# Autodesk Inventor assembly: CC2x2
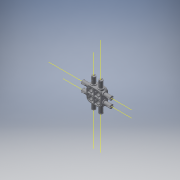
[picture p0: Inventor's stored thumbnail of the model, 180x180]
Saved by Autodesk Inventor 2019.3 (Build 233278000, 278)
## iProperties
Created: 2019-02-06
Part Number: CC2x2
Document SubType Name: Assembly
Designer: Varga Daniel
Author: Varga Daniel
## Documents named in this file (5)
- C:\!_Dani\!_cloud\OneDrive\!_munka\Revolution\RevvyDemoKit\Structural parts\Connector Boxes\Connector cubes\CC2x2_X.iam
- C:\!_Dani\!_cloud\OneDrive\!_munka\Revolution\RevvyDemoKit\Structural parts\Connector Boxes\Connector_box_L_base.ipt
- C:\!_Dani\!_cloud\OneDrive\!_munka\Revolution\RevvyDemoKit\Structural parts\Connector Boxes\Connector_box_collar\Connector_box_collar-one_side.ipt
- C:\!_Dani\!_cloud\OneDrive\!_munka\Revolution\RevvyDemoKit\Structural parts\Connector Boxes\Connector_box_collar.ipt
- C:\!_Dani\!_cloud\OneDrive\!_munka\Revolution\RevvyDemoKit\Structural parts\Connetor Pins\Connector_pin_stick.ipt
## Components (20 placed, 3 different names)
1. Connector_box_L_base:1 — Flush:1, Flush:2, Mate:41, Flush:3, Flush:4, Mate:42, Mate:54, Mate:55, Angle:6, Mate:56, Mate:57, Angle:7
2. Connector_box_collar-one_side:1 — Mate:7, Mate:8, Mate:57
3. Connector_box_collar-one_side:2 — Mate:9, Mate:10, Mate:55
4. Connector_pin_stick:1 — Mate:7, Mate:8, Mate:56, Angle:7
5. Connector_pin_stick:2 — Mate:9, Mate:10, Mate:54, Angle:6
6. Connector_box_collar-one_side:3 — Mate:47
7. Connector_box_collar-one_side:4 — Mate:49
8. Connector_pin_stick:3 — Mate:46, Angle:2
9. Connector_pin_stick:4 — Mate:48, Angle:3
10. Connector_box_collar-one_side:5 — Mate:51
11. Connector_box_collar-one_side:6 — Mate:53
12. Connector_pin_stick:5 — Mate:50, Angle:4
13. Connector_pin_stick:6 — Mate:52, Angle:5
14. Connector_box_collar-one_side:7 — Mate:45
15. Connector_box_collar-one_side:8 — Mate:59
16. Connector_pin_stick:7 — Mate:44, Angle:1
17. Connector_pin_stick:8 — Mate:58, Angle:8
18. Connector_box_L_base:6 — Flush:1, Flush:2, Mate:41, Flush:5, Flush:6, Mate:43, Mate:44, Mate:45, Angle:1, Mate:58, Mate:59, Angle:8
19. Connector_box_L_base:7 — Flush:3, Flush:4, Mate:42, Mate:50, Mate:51, Angle:4, Mate:52, Mate:53, Angle:5
20. Connector_box_L_base:8 — Flush:5, Flush:6, Mate:43, Mate:46, Mate:47, Angle:2, Mate:48, Mate:49, Angle:3
## Relationships (49: Mate 35, Angle 8, Flush 6)
- Mate:7: Connector_box_collar-one_side:1 ↔ Connector_pin_stick:1
- Mate:8: Connector_box_collar-one_side:1 ↔ Connector_pin_stick:1
- Mate:9: Connector_box_collar-one_side:2 ↔ Connector_pin_stick:2
- Mate:10: Connector_box_collar-one_side:2 ↔ Connector_pin_stick:2
- [Mate]: Connector_box_collar-one_side:3 ↔ Connector_pin_stick:3
- [Mate]: Connector_box_collar-one_side:3 ↔ Connector_pin_stick:3
- [Mate]: Connector_box_collar-one_side:4 ↔ Connector_pin_stick:4
- [Mate]: Connector_box_collar-one_side:4 ↔ Connector_pin_stick:4
- [Mate]: Connector_box_collar-one_side:5 ↔ Connector_pin_stick:5
- [Mate]: Connector_box_collar-one_side:5 ↔ Connector_pin_stick:5
- [Mate]: Connector_box_collar-one_side:6 ↔ Connector_pin_stick:6
- [Mate]: Connector_box_collar-one_side:6 ↔ Connector_pin_stick:6
- [Mate]: Connector_box_collar-one_side:7 ↔ Connector_pin_stick:7
- [Mate]: Connector_box_collar-one_side:7 ↔ Connector_pin_stick:7
- [Mate]: Connector_box_collar-one_side:8 ↔ Connector_pin_stick:8
- [Mate]: Connector_box_collar-one_side:8 ↔ Connector_pin_stick:8
- Flush:1: Connector_box_L_base:1 ↔ Connector_box_L_base:6
- Flush:2: Connector_box_L_base:1 ↔ Connector_box_L_base:6
- Mate:41: Connector_box_L_base:1 ↔ Connector_box_L_base:6
- Flush:3: Connector_box_L_base:1 ↔ Connector_box_L_base:7
- Flush:4: Connector_box_L_base:1 ↔ Connector_box_L_base:7
- Mate:42: Connector_box_L_base:1 ↔ Connector_box_L_base:7
- Flush:5: Connector_box_L_base:6 ↔ Connector_box_L_base:8
- Flush:6: Connector_box_L_base:6 ↔ Connector_box_L_base:8
- Mate:43: Connector_box_L_base:6 ↔ Connector_box_L_base:8
- Mate:44: Connector_pin_stick:7 ↔ Connector_box_L_base:6
- Mate:45: Connector_box_collar-one_side:7 ↔ Connector_box_L_base:6
- Angle:1 (0 deg): Connector_pin_stick:7 ↔ Connector_box_L_base:6
- Mate:46: Connector_pin_stick:3 ↔ Connector_box_L_base:8
- Mate:47: Connector_box_collar-one_side:3 ↔ Connector_box_L_base:8
- Angle:2 (0 deg): Connector_pin_stick:3 ↔ Connector_box_L_base:8
- Mate:48: Connector_pin_stick:4 ↔ Connector_box_L_base:8
- Mate:49: Connector_box_collar-one_side:4 ↔ Connector_box_L_base:8
- Angle:3 (0 deg): Connector_pin_stick:4 ↔ Connector_box_L_base:8
- Mate:50: Connector_pin_stick:5 ↔ Connector_box_L_base:7
- Mate:51: Connector_box_collar-one_side:5 ↔ Connector_box_L_base:7
- Angle:4 (0 deg): Connector_pin_stick:5 ↔ Connector_box_L_base:7
- Mate:52: Connector_pin_stick:6 ↔ Connector_box_L_base:7
- Mate:53: Connector_box_collar-one_side:6 ↔ Connector_box_L_base:7
- Angle:5 (0 deg): Connector_pin_stick:6 ↔ Connector_box_L_base:7
- Mate:54: Connector_box_L_base:1 ↔ Connector_pin_stick:2
- Mate:55: Connector_box_L_base:1 ↔ Connector_box_collar-one_side:2
- Angle:6 (0 deg): Connector_box_L_base:1 ↔ Connector_pin_stick:2
- Mate:56: Connector_box_L_base:1 ↔ Connector_pin_stick:1
- Mate:57: Connector_box_L_base:1 ↔ Connector_box_collar-one_side:1
- Angle:7 (0 deg): Connector_box_L_base:1 ↔ Connector_pin_stick:1
- Mate:58: Connector_pin_stick:8 ↔ Connector_box_L_base:6
- Mate:59: Connector_box_collar-one_side:8 ↔ Connector_box_L_base:6
- Angle:8 (0 deg): Connector_pin_stick:8 ↔ Connector_box_L_base:6
## Named parameters: d18_d6 = 0 mm, d19_d7 = 0 mm, d20_d8 = 0 mm, d21_d9 = 0 mm, d30_d6 = 0 mm, d31_d7 = 0 mm, d32_d8 = 0 mm, d33_d9 = 0 mm, d42_d6 = 0 mm, d43_d7 = 0 mm, d44_d8 = 0 mm, d45_d9 = 0 mm, Inner_thickness = 1 mm, Hole_height = 8.4 mm
